# Autodesk Inventor assembly: assembly
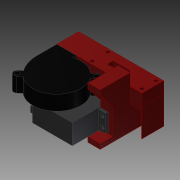
[picture p0: Inventor's stored thumbnail of the model, 180x180]
Saved by Autodesk Inventor 2013 (Build 170138000, 138)
## iProperties
Created: 2014-04-23
Part Number: assembly
Document SubType Name: Assembly
Designer: Masta
Author: Masta
## Documents named in this file (12)
- D:\DrOctopus\3D model\extruder\extruder.iam
- D:\DrOctopus\3D model\extruder\servo HK15138.ipt
- D:\DrOctopus\3D model\extruder\servo arm.ipt
- D:\DrOctopus\3D model\extruder\adapter.ipt
- D:\DrOctopus\3D model\extruder\tulejka M2x4.ipt
- C:\Users\Masta\Documents\Inventor\Content Center Files\R2013\en-US\DIN 7985 (H)\DIN 7985 (H) - M5x30-H.ipt
- C:\Users\Masta\Documents\Inventor\Content Center Files\R2013\en-US\DIN 934\DIN 934 - M5 x 0.8.ipt
- D:\DrOctopus\3D model\extruder\MK7 gear.ipt
- D:\DrOctopus\3D model\extruder\body.ipt
- C:\Users\Masta\Documents\Inventor\Content Center Files\R2013\en-US\DIN BEARING(1)\DIN 625 SKF - SKF 625.ipt
- D:\DrOctopus\3D model\extruder\grip.ipt
- D:\DrOctopus\3D model\extruder\fan.ipt
## Components (13 placed, 11 different names)
1. servo HK15138:1 — Insert:1, Flush:1, Flush:3
2. servo arm:1 — Insert:1, Insert:2, Insert:3
3. adapter:1 — Insert:4, Insert:5, Insert:6, Insert:10
4. tulejka M2x4:1 — Insert:2, Insert:4
5. tulejka M2x4:2 — Insert:3, Insert:5
6. DIN 7985 (H) M5x30-H:1 — Insert:6, Mate:2
7. MK7 gear:1 — Insert:10, Insert:11
8. DIN 934 - replaced by DIN EN 24032/28673/28674 M5:3 — Insert:9
9. DIN 625 SKF 625:1 — Insert:9, Insert:11
10. body:1 — Flush:1, Angle:3, Flush:3, Flush:4, Flush:5, Mate:3, Mate:4, Mate:5, Mate:6
11. DIN 625 SKF 625:2 — Insert:12
12. grip:1 — Flush:4, Flush:5, Insert:12, Mate:3, Mate:4, Mate:7
13. fan:1 — Mate:5, Mate:6, Mate:7
## Relationships (21: Insert 10, Mate 6, Flush 4, Angle 1)
- Insert:1: servo HK15138:1 ↔ servo arm:1
- Insert:2: servo arm:1 ↔ tulejka M2x4:1
- Insert:3: servo arm:1 ↔ tulejka M2x4:2
- Insert:4: adapter:1 ↔ tulejka M2x4:1
- Insert:5: adapter:1 ↔ tulejka M2x4:2
- Insert:6: adapter:1 ↔ DIN 7985 (H) M5x30-H:1
- Insert:9: DIN 934 - replaced by DIN EN 24032/28673/28674 M5:3 ↔ DIN 625 SKF 625:1
- Flush:1: servo HK15138:1 ↔ body:1
- Mate:2: DIN 7985 (H) M5x30-H:1
- Angle:3 (90 deg): body:1
- Insert:10: adapter:1 ↔ MK7 gear:1
- Insert:11: MK7 gear:1 ↔ DIN 625 SKF 625:1
- Flush:3: servo HK15138:1 ↔ body:1
- Flush:4: body:1 ↔ grip:1
- Flush:5: body:1 ↔ grip:1
- Insert:12 (0.5 mm): DIN 625 SKF 625:2 ↔ grip:1
- Mate:3: body:1 ↔ grip:1
- Mate:4: body:1 ↔ grip:1
- Mate:5: body:1 ↔ fan:1
- Mate:6: body:1 ↔ fan:1
- Mate:7: grip:1 ↔ fan:1
